# Autodesk Inventor assembly: Radiator samling
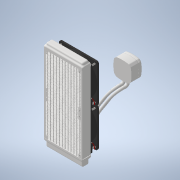
[picture p0: Inventor's stored thumbnail of the model, 180x180]
Saved by Autodesk Inventor 2020 (Build 240168000, 168)
## iProperties
Created: 2021-05-19
Part Number: Radiator samling
Document SubType Name: Assembly
Designer: 6128059
Author: 6128059
## Documents named in this file (12)
- C:\Users\6128059\OneDrive - Roskilde Tekniske Skole\SKP\Inventor\PC\Radiator samling.iam
- C:\Users\6128059\OneDrive - Roskilde Tekniske Skole\SKP\Inventor\PC\Kølerør.ipt
- C:\Users\6128059\OneDrive - Roskilde Tekniske Skole\SKP\Inventor\PC\Gitter.ipt
- C:\Users\6128059\OneDrive - Roskilde Tekniske Skole\SKP\Inventor\PC\Yderskal - Sheet metal.ipt
- C:\Users\6128059\OneDrive - Roskilde Tekniske Skole\SKP\Inventor\PC\Radiator - Lukket ende.ipt
- C:\Users\6128059\OneDrive - Roskilde Tekniske Skole\SKP\Inventor\PC\Radiator - Åben ende.ipt
- C:\Users\6128059\OneDrive - Roskilde Tekniske Skole\SKP\Inventor\PC\120 mm fan assembly.iam
- C:\Users\6128059\OneDrive - Roskilde Tekniske Skole\SKP\Inventor\PC\Water block.ipt
- C:\Users\6128059\OneDrive - Roskilde Tekniske Skole\SKP\Inventor\PC\Rørende.ipt
- C:\Users\6128059\OneDrive - Roskilde Tekniske Skole\SKP\Inventor\PC\Rørende - water block.ipt
- C:\Users\6128059\OneDrive - Roskilde Tekniske Skole\SKP\Inventor\PC\Rør 1.ipt
- C:\Users\6128059\OneDrive - Roskilde Tekniske Skole\SKP\Inventor\PC\ANSI B18.6.7M - M5x0,8 x 30(5).ipt
## Components (35 placed, 11 different names)
1. Kølerør:1 — Tangent:1, Mate:1, Tangent:2, Flush:1, Mate:11, Mate:12, Flush:2, Mate:13, Flush:3, Flush:4, Mate:14
2. Yderskal - Sheet metal:1 — Mate:8, Mate:9, Mate:10, Mate:11
3. Yderskal - Sheet metal:2 — Mate:2, Mate:3, Mate:4, Mate:5, Mate:6, Mate:7, Mate:12, Flush:2
4. 120 mm fan assembly:1 [sub-assembly] — Mate:2, Mate:3, Mate:4, Mate:10, Mate:17, Mate:32, Mate:33
5. 120 mm fan assembly:2 [sub-assembly] — Mate:5, Mate:6, Mate:7, Mate:8, Mate:9, Mate:30, Mate:31
6. Radiator - Åben ende:1 — Mate:13, Flush:3, Flush:4, Mate:15, Mate:16, Flush:5, Flush:6, Mate:20, Mate:21, Mate:22, Mate:23
7. Radiator - Lukket ende:1 — Mate:14, Mate:15, Mate:16
8. Water block:1 — Flush:5, Mate:17, Flush:6, Mate:24, Mate:25, Mate:26, Mate:27
9. Rørende:3 — Mate:21, Mate:22, Flush:7
10. Rørende:4 — Mate:20, Mate:23
11. Rørende - water block:1 — Mate:25, Mate:27, Angle:1, Mate:28, Mate:29
12. Rørende - water block:2 — Mate:24, Mate:26, Angle:1, Flush:8
13. Rør 1:1 — Flush:7, Flush:8
14. Rør 1:2 — Mate:28, Mate:29
15. Gitter:1 — Tangent:1, Mate:1, Tangent:2, Flush:1
16. Gitter:2
17. Gitter:3
18. Gitter:4
19. Gitter:5
20. Gitter:6
21. Gitter:7
22. Gitter:8
23. Gitter:9
24. Gitter:10
25. Gitter:11
26. Gitter:12
27. Gitter:13
28. Cross Recessed Pan Head Machine Screw - Type IA - Metric M5x0,8 x 30:1 — Mate:30, Mate:31
29. Cross Recessed Pan Head Machine Screw - Type IA - Metric M5x0,8 x 30:2
30. Cross Recessed Pan Head Machine Screw - Type IA - Metric M5x0,8 x 30:3
31. Cross Recessed Pan Head Machine Screw - Type IA - Metric M5x0,8 x 30:4
32. Cross Recessed Pan Head Machine Screw - Type IA - Metric M5x0,8 x 30:5 — Mate:32, Mate:33
33. Cross Recessed Pan Head Machine Screw - Type IA - Metric M5x0,8 x 30:6
34. Cross Recessed Pan Head Machine Screw - Type IA - Metric M5x0,8 x 30:7
35. Cross Recessed Pan Head Machine Screw - Type IA - Metric M5x0,8 x 30:8
## Component patterns: (13 elements, first: Gitter:1), (4 elements, first: Cross Recessed Pan Head Machine Screw - Type IA - Metric M5x0,8 x 30:1), (4 elements, first: Cross Recessed Pan Head Machine Screw - Type IA - Metric M5x0,8 x 30:5)
## Relationships (42: Mate 31, Flush 8, Tangent 2, Angle 1)
- Tangent:1: Kølerør:1 ↔ Gitter:1
- Mate:1: Kølerør:1 ↔ Gitter:1
- Tangent:2: Kølerør:1 ↔ Gitter:1
- Flush:1: Kølerør:1 ↔ Gitter:1
- Mate:2: Yderskal - Sheet metal:2 ↔ 120 mm fan assembly:1
- Mate:3: Yderskal - Sheet metal:2 ↔ 120 mm fan assembly:1
- Mate:4: Yderskal - Sheet metal:2 ↔ 120 mm fan assembly:1
- Mate:5: Yderskal - Sheet metal:2 ↔ 120 mm fan assembly:2
- Mate:6: Yderskal - Sheet metal:2 ↔ 120 mm fan assembly:2
- Mate:7: Yderskal - Sheet metal:2 ↔ 120 mm fan assembly:2
- Mate:8: Yderskal - Sheet metal:1 ↔ 120 mm fan assembly:2
- Mate:9: Yderskal - Sheet metal:1 ↔ 120 mm fan assembly:2
- Mate:10: Yderskal - Sheet metal:1 ↔ 120 mm fan assembly:1
- Mate:11: Kølerør:1 ↔ Yderskal - Sheet metal:1
- Mate:12: Kølerør:1 ↔ Yderskal - Sheet metal:2
- Flush:2: Kølerør:1 ↔ Yderskal - Sheet metal:2
- Mate:13: Kølerør:1 ↔ Radiator - Åben ende:1
- Flush:3: Kølerør:1 ↔ Radiator - Åben ende:1
- Flush:4: Kølerør:1 ↔ Radiator - Åben ende:1
- Mate:14: Kølerør:1 ↔ Radiator - Lukket ende:1
- Mate:15: Radiator - Åben ende:1 ↔ Radiator - Lukket ende:1
- Mate:16: Radiator - Åben ende:1 ↔ Radiator - Lukket ende:1
- Flush:5: Radiator - Åben ende:1 ↔ Water block:1
- Mate:17 (100 mm): 120 mm fan assembly:1 ↔ Water block:1
- Flush:6 (150 mm): Radiator - Åben ende:1 ↔ Water block:1
- Mate:20: Radiator - Åben ende:1 ↔ Rørende:4
- Mate:21: Radiator - Åben ende:1 ↔ Rørende:3
- Mate:22 (5 mm): Radiator - Åben ende:1 ↔ Rørende:3
- Mate:23 (5 mm): Radiator - Åben ende:1 ↔ Rørende:4
- Mate:24: Water block:1 ↔ Rørende - water block:2
- Mate:25: Water block:1 ↔ Rørende - water block:1
- Mate:26: Water block:1 ↔ Rørende - water block:2
- Mate:27: Water block:1 ↔ Rørende - water block:1
- Angle:1 (0 deg): Rørende - water block:1 ↔ Rørende - water block:2
- Flush:7: Rørende:3 ↔ Rør 1:1
- Flush:8: Rørende - water block:2 ↔ Rør 1:1
- Mate:28: Rørende - water block:1 ↔ Rør 1:2
- Mate:29: Rørende - water block:1 ↔ Rør 1:2
- Mate:30: 120 mm fan assembly:2 ↔ Cross Recessed Pan Head Machine Screw - Type IA - Metric M5x0,8 x 30:1
- Mate:31: 120 mm fan assembly:2 ↔ Cross Recessed Pan Head Machine Screw - Type IA - Metric M5x0,8 x 30:1
- Mate:32: 120 mm fan assembly:1 ↔ Cross Recessed Pan Head Machine Screw - Type IA - Metric M5x0,8 x 30:5
- Mate:33: 120 mm fan assembly:1 ↔ Cross Recessed Pan Head Machine Screw - Type IA - Metric M5x0,8 x 30:5
